# Autodesk Inventor assembly: Estrutura de perfis_999
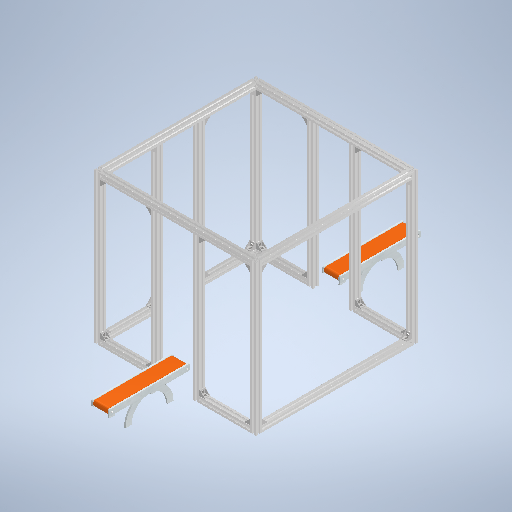
[picture p0: Inventor's stored thumbnail of the model, 512x512]
Saved by Autodesk Inventor 2026 (Build 300175000, 175)
## iProperties
Created: 2025-05-20
Part Number: Estrutura de perfis_999
Document SubType Name: Assembly
Designer: carlo
Author: carlo
## Documents named in this file (11)
- C:\Users\carlo\Documents\Projeto - Braco Robotico\Design\Estrutura de perfis\Estrutura de perfis_999.iam
- C:\Users\carlo\Documents\Projeto - Braco Robotico\Design\Estrutura de perfis\perfil_20x20_001.ipt
- C:\Users\carlo\Documents\Projeto - Braco Robotico\Design\Estrutura de perfis\perfil_20x20_002.ipt
- C:\Users\carlo\Documents\Projeto - Braco Robotico\Design\Estrutura de perfis\perfil_20x20_003.ipt
- C:\Users\carlo\Documents\Projeto - Braco Robotico\Design\Estrutura de perfis\perfil_20x20_004.ipt
- C:\Users\carlo\Documents\Projeto - Braco Robotico\Design\Estrutura de perfis\CBR2020\CBR2020\CBR2020.ipt
- C:\Users\carlo\Documents\Projeto - Braco Robotico\Design\Estrutura de perfis\BPN06M4\BPN06M4\BPN06M4.ipt
- C:\Users\carlo\Documents\Inventor\Content Center Files\R2026\en-US\BS 4183(4)\BS 4183 - M4 x 8(1) III.ipt
- C:\Users\carlo\Documents\Projeto - Braco Robotico\Design\Estrutura de perfis\Conveyor_001_001.ipt
- C:\Users\carlo\Documents\Projeto - Braco Robotico\Design\Estrutura de perfis\Conveyor_002_001.ipt
- C:\Users\carlo\Documents\Projeto - Braco Robotico\Design\Estrutura de perfis\Conveyor_003_001.ipt
## Components (169 placed, 10 different names)
1. perfil_20x20_001:1 — Flush:6, Mate:4, Flush:10
2. perfil_20x20_001:3 — Flush:13, Mate:6, Flush:14, Mate:8, Flush:39, Flush:62
3. perfil_20x20_001:4 — Flush:4, Mate:1, Flush:8, Mate:3, Flush:9, Flush:32
4. perfil_20x20_002:1 — Flush:4, Mate:1, Flush:6, Mate:30
5. perfil_20x20_002:3 — Flush:8, Mate:3, Flush:9, Mate:4, Flush:10, Flush:11, Mate:5, Flush:12, Flush:13, Mate:6, Flush:14, Mate:34, Flush:49, Mate:35, Flush:51
6. perfil_20x20_003:1 — Flush:11, Mate:5, Flush:12, Flush:15, Mate:7, Flush:16, Mate:33, Mate:38
7. perfil_20x20_004:1 — Flush:15, Mate:7, Flush:16, Flush:17, Symmetry:1, Flush:48, Flush:63, Flush:64
8. perfil_20x20_004:2 — Flush:17, Mate:8, Symmetry:1, Flush:18, Mate:9, Flush:19
9. perfil_20x20_003:2 — Flush:18, Mate:9, Flush:19, Flush:20, Mate:10, Flush:21
10. perfil_20x20_002:4 — Flush:20, Mate:10, Flush:21, Flush:22, Mate:11, Flush:23, Flush:24, Flush:31, Mate:23
11. perfil_20x20_001:5 — Flush:22, Mate:11, Flush:23, Mate:12, Flush:25, Mate:25
12. perfil_20x20_002:5 — Flush:24, Mate:12, Flush:25, Mate:24, Flush:38, Mate:28, Flush:40, Mate:29, Flush:44
13. perfil_20x20_003:3 — Flush:31, Flush:32, Mate:23, Flush:33, Flush:34, Flush:35, Mate:26
14. perfil_20x20_003:4 — Flush:33, Mate:24, Flush:34, Mate:27, Flush:41
15. perfil_20x20_004:3 — Flush:35, Mate:25, Mate:26, Flush:36, Flush:37
16. perfil_20x20_004:4 — Flush:36, Flush:37, Mate:27, Flush:45
17. perfil_20x20_001:6 — Flush:38, Flush:39, Mate:28, Flush:57
18. perfil_20x20_003:5 — Flush:40, Flush:41, Mate:29, Flush:42, Flush:43, Mate:31
19. perfil_20x20_003:6 — Flush:42, Flush:43, Mate:30, Mate:32
20. perfil_20x20_004:5 — Flush:44, Flush:45, Mate:31, Flush:46, Flush:47
21. perfil_20x20_004:6 — Flush:46, Flush:47, Mate:32, Flush:58, Flush:59
22. CBR2020:17
23. BPN06M4:33
24. BS 4183 Specification for machine screws and machine screw nuts. Metric series - Metric M4 x 8:33
25. BPN06M4:34
26. BS 4183 Specification for machine screws and machine screw nuts. Metric series - Metric M4 x 8:34
27. CBR2020:18
28. BPN06M4:35
29. BS 4183 Specification for machine screws and machine screw nuts. Metric series - Metric M4 x 8:35
30. BPN06M4:36
31. BS 4183 Specification for machine screws and machine screw nuts. Metric series - Metric M4 x 8:36
32. CBR2020:19
33. BPN06M4:37
34. BS 4183 Specification for machine screws and machine screw nuts. Metric series - Metric M4 x 8:37
35. BPN06M4:38
36. BS 4183 Specification for machine screws and machine screw nuts. Metric series - Metric M4 x 8:38
37. CBR2020:20
38. BPN06M4:39
39. BS 4183 Specification for machine screws and machine screw nuts. Metric series - Metric M4 x 8:39
40. BPN06M4:40
41. BS 4183 Specification for machine screws and machine screw nuts. Metric series - Metric M4 x 8:40
42. CBR2020:21
43. BPN06M4:41
44. BS 4183 Specification for machine screws and machine screw nuts. Metric series - Metric M4 x 8:41
45. BPN06M4:42
46. BS 4183 Specification for machine screws and machine screw nuts. Metric series - Metric M4 x 8:42
47. CBR2020:22
48. BPN06M4:43
49. BS 4183 Specification for machine screws and machine screw nuts. Metric series - Metric M4 x 8:43
50. BPN06M4:44
51. BS 4183 Specification for machine screws and machine screw nuts. Metric series - Metric M4 x 8:44
52. CBR2020:23
53. BPN06M4:45
54. BS 4183 Specification for machine screws and machine screw nuts. Metric series - Metric M4 x 8:45
55. BPN06M4:46
56. BS 4183 Specification for machine screws and machine screw nuts. Metric series - Metric M4 x 8:46
57. CBR2020:24
58. BPN06M4:47
59. BS 4183 Specification for machine screws and machine screw nuts. Metric series - Metric M4 x 8:47
60. BPN06M4:48
61. BS 4183 Specification for machine screws and machine screw nuts. Metric series - Metric M4 x 8:48
62. CBR2020:25
63. BPN06M4:49
64. BS 4183 Specification for machine screws and machine screw nuts. Metric series - Metric M4 x 8:49
65. BPN06M4:50
66. BS 4183 Specification for machine screws and machine screw nuts. Metric series - Metric M4 x 8:50
67. CBR2020:26
68. BPN06M4:51
69. BS 4183 Specification for machine screws and machine screw nuts. Metric series - Metric M4 x 8:51
70. BPN06M4:52
71. BS 4183 Specification for machine screws and machine screw nuts. Metric series - Metric M4 x 8:52
72. CBR2020:27
73. BPN06M4:53
74. BS 4183 Specification for machine screws and machine screw nuts. Metric series - Metric M4 x 8:53
75. BPN06M4:54
76. BS 4183 Specification for machine screws and machine screw nuts. Metric series - Metric M4 x 8:54
77. CBR2020:28
78. BPN06M4:55
79. BS 4183 Specification for machine screws and machine screw nuts. Metric series - Metric M4 x 8:55
80. BPN06M4:56
81. BS 4183 Specification for machine screws and machine screw nuts. Metric series - Metric M4 x 8:56
82. CBR2020:9
83. BPN06M4:17
84. BS 4183 Specification for machine screws and machine screw nuts. Metric series - Metric M4 x 8:17
85. BPN06M4:18
86. BS 4183 Specification for machine screws and machine screw nuts. Metric series - Metric M4 x 8:18
87. CBR2020:10
88. BPN06M4:19
89. BS 4183 Specification for machine screws and machine screw nuts. Metric series - Metric M4 x 8:19
90. BPN06M4:20
91. BS 4183 Specification for machine screws and machine screw nuts. Metric series - Metric M4 x 8:20
92. CBR2020:11
93. BPN06M4:21
94. BS 4183 Specification for machine screws and machine screw nuts. Metric series - Metric M4 x 8:21
95. BPN06M4:22
96. BS 4183 Specification for machine screws and machine screw nuts. Metric series - Metric M4 x 8:22
97. CBR2020:12
98. BPN06M4:23
99. BS 4183 Specification for machine screws and machine screw nuts. Metric series - Metric M4 x 8:23
100. BPN06M4:24
101. BS 4183 Specification for machine screws and machine screw nuts. Metric series - Metric M4 x 8:24
102. CBR2020:13
103. BPN06M4:25
104. BS 4183 Specification for machine screws and machine screw nuts. Metric series - Metric M4 x 8:25
105. BPN06M4:26
106. BS 4183 Specification for machine screws and machine screw nuts. Metric series - Metric M4 x 8:26
107. CBR2020:14
108. BPN06M4:27
109. BS 4183 Specification for machine screws and machine screw nuts. Metric series - Metric M4 x 8:27
110. BPN06M4:28
111. BS 4183 Specification for machine screws and machine screw nuts. Metric series - Metric M4 x 8:28
112. CBR2020:15
113. BPN06M4:29
114. BS 4183 Specification for machine screws and machine screw nuts. Metric series - Metric M4 x 8:29
115. BPN06M4:30
116. BS 4183 Specification for machine screws and machine screw nuts. Metric series - Metric M4 x 8:30
117. CBR2020:16
118. BPN06M4:31
119. BS 4183 Specification for machine screws and machine screw nuts. Metric series - Metric M4 x 8:31
120. BPN06M4:32
121. BS 4183 Specification for machine screws and machine screw nuts. Metric series - Metric M4 x 8:32
122. CBR2020:5
123. BPN06M4:9
124. BS 4183 Specification for machine screws and machine screw nuts. Metric series - Metric M4 x 8:9
125. BPN06M4:10
126. BS 4183 Specification for machine screws and machine screw nuts. Metric series - Metric M4 x 8:10
127. CBR2020:6
128. BPN06M4:11
129. BS 4183 Specification for machine screws and machine screw nuts. Metric series - Metric M4 x 8:11
130. BPN06M4:12
131. BS 4183 Specification for machine screws and machine screw nuts. Metric series - Metric M4 x 8:12
132. CBR2020:7
133. BPN06M4:13
134. BS 4183 Specification for machine screws and machine screw nuts. Metric series - Metric M4 x 8:13
135. BPN06M4:14
136. BS 4183 Specification for machine screws and machine screw nuts. Metric series - Metric M4 x 8:14
137. CBR2020:8
138. BPN06M4:15
139. BS 4183 Specification for machine screws and machine screw nuts. Metric series - Metric M4 x 8:15
140. BPN06M4:16
141. BS 4183 Specification for machine screws and machine screw nuts. Metric series - Metric M4 x 8:16
142. CBR2020:3
143. BPN06M4:5
144. BS 4183 Specification for machine screws and machine screw nuts. Metric series - Metric M4 x 8:5
145. BPN06M4:6
146. BS 4183 Specification for machine screws and machine screw nuts. Metric series - Metric M4 x 8:6
147. CBR2020:4
148. BPN06M4:7
149. BS 4183 Specification for machine screws and machine screw nuts. Metric series - Metric M4 x 8:7
150. BPN06M4:8
151. BS 4183 Specification for machine screws and machine screw nuts. Metric series - Metric M4 x 8:8
152. CBR2020:2
153. BPN06M4:3
154. BS 4183 Specification for machine screws and machine screw nuts. Metric series - Metric M4 x 8:3
155. BPN06M4:4
156. BS 4183 Specification for machine screws and machine screw nuts. Metric series - Metric M4 x 8:4
157. BS 4183 Specification for machine screws and machine screw nuts. Metric series - Metric M4 x 8:2 — Mate:39, Mate:40
158. BPN06M4:2 — Flush:51, Mate:38, Flush:52, Mate:39
159. BS 4183 Specification for machine screws and machine screw nuts. Metric series - Metric M4 x 8:1 — Mate:36, Mate:37
160. BPN06M4:1 — Flush:49, Mate:35, Flush:50, Mate:36
161. CBR2020:1 — Flush:48, Mate:33, Mate:34, Flush:50, Mate:37, Flush:52, Mate:40
162. Conveyor_003_001:1 — Mate:43, Mate:44, Mate:49
163. Conveyor_002_001:2 — Mate:42, Flush:54, Mate:49
164. Conveyor_002_001:1 — Mate:41, Flush:53, Mate:43
165. Conveyor_001_001:1 — Mate:41, Flush:53, Mate:42, Flush:54, Mate:44, Flush:57, Flush:58, Flush:59
166. Conveyor_001_001:2 — Flush:62, Flush:63, Flush:64
167. Conveyor_002_001:3
168. Conveyor_002_001:4
169. Conveyor_003_001:2
## Relationships (92: Flush 52, Mate 39, Symmetry 1)
- Flush:4: perfil_20x20_001:4 ↔ perfil_20x20_002:1
- Mate:1: perfil_20x20_001:4 ↔ perfil_20x20_002:1
- Flush:6: perfil_20x20_001:1 ↔ perfil_20x20_002:1
- Flush:8: perfil_20x20_001:4 ↔ perfil_20x20_002:3
- Mate:3: perfil_20x20_001:4 ↔ perfil_20x20_002:3
- Flush:9: perfil_20x20_001:4 ↔ perfil_20x20_002:3
- Mate:4: perfil_20x20_001:1 ↔ perfil_20x20_002:3
- Flush:10: perfil_20x20_001:1 ↔ perfil_20x20_002:3
- Flush:11: perfil_20x20_002:3 ↔ perfil_20x20_003:1
- Mate:5: perfil_20x20_002:3 ↔ perfil_20x20_003:1
- Flush:12: perfil_20x20_002:3 ↔ perfil_20x20_003:1
- Flush:13: perfil_20x20_001:3 ↔ perfil_20x20_002:3
- Mate:6: perfil_20x20_001:3 ↔ perfil_20x20_002:3
- Flush:14: perfil_20x20_001:3 ↔ perfil_20x20_002:3
- Flush:15: perfil_20x20_003:1 ↔ perfil_20x20_004:1
- Mate:7: perfil_20x20_003:1 ↔ perfil_20x20_004:1
- Flush:16: perfil_20x20_003:1 ↔ perfil_20x20_004:1
- Flush:17: perfil_20x20_004:1 ↔ perfil_20x20_004:2
- Mate:8: perfil_20x20_001:3 ↔ perfil_20x20_004:2
- Symmetry:1: perfil_20x20_004:1 ↔ perfil_20x20_004:2
- Flush:18: perfil_20x20_004:2 ↔ perfil_20x20_003:2
- Mate:9: perfil_20x20_004:2 ↔ perfil_20x20_003:2
- Flush:19: perfil_20x20_004:2 ↔ perfil_20x20_003:2
- Flush:20: perfil_20x20_003:2 ↔ perfil_20x20_002:4
- Mate:10: perfil_20x20_003:2 ↔ perfil_20x20_002:4
- Flush:21: perfil_20x20_003:2 ↔ perfil_20x20_002:4
- Flush:22: perfil_20x20_002:4 ↔ perfil_20x20_001:5
- Mate:11: perfil_20x20_002:4 ↔ perfil_20x20_001:5
- Flush:23: perfil_20x20_002:4 ↔ perfil_20x20_001:5
- Flush:24: perfil_20x20_002:4 ↔ perfil_20x20_002:5
- Mate:12: perfil_20x20_001:5 ↔ perfil_20x20_002:5
- Flush:25: perfil_20x20_001:5 ↔ perfil_20x20_002:5
- Flush:31: perfil_20x20_002:4 ↔ perfil_20x20_003:3
- Flush:32: perfil_20x20_001:4 ↔ perfil_20x20_003:3
- Mate:23: perfil_20x20_002:4 ↔ perfil_20x20_003:3
- Flush:33: perfil_20x20_003:3 ↔ perfil_20x20_003:4
- Mate:24: perfil_20x20_002:5 ↔ perfil_20x20_003:4
- Flush:34: perfil_20x20_003:3 ↔ perfil_20x20_003:4
- Flush:35: perfil_20x20_003:3 ↔ perfil_20x20_004:3
- Mate:25: perfil_20x20_001:5 ↔ perfil_20x20_004:3
- Mate:26: perfil_20x20_003:3 ↔ perfil_20x20_004:3
- Flush:36: perfil_20x20_004:3 ↔ perfil_20x20_004:4
- Flush:37: perfil_20x20_004:3 ↔ perfil_20x20_004:4
- Mate:27: perfil_20x20_003:4 ↔ perfil_20x20_004:4
- Flush:38: perfil_20x20_002:5 ↔ perfil_20x20_001:6
- Flush:39: perfil_20x20_001:3 ↔ perfil_20x20_001:6
- Mate:28: perfil_20x20_002:5 ↔ perfil_20x20_001:6
- Flush:40: perfil_20x20_002:5 ↔ perfil_20x20_003:5
- Flush:41: perfil_20x20_003:4 ↔ perfil_20x20_003:5
- Mate:29: perfil_20x20_002:5 ↔ perfil_20x20_003:5
- Flush:42: perfil_20x20_003:5 ↔ perfil_20x20_003:6
- Flush:43: perfil_20x20_003:5 ↔ perfil_20x20_003:6
- Mate:30: perfil_20x20_002:1 ↔ perfil_20x20_003:6
- Flush:44: perfil_20x20_002:5 ↔ perfil_20x20_004:5
- Flush:45: perfil_20x20_004:4 ↔ perfil_20x20_004:5
- Mate:31: perfil_20x20_003:5 ↔ perfil_20x20_004:5
- Flush:46: perfil_20x20_004:5 ↔ perfil_20x20_004:6
- Flush:47: perfil_20x20_004:5 ↔ perfil_20x20_004:6
- Mate:32: perfil_20x20_003:6 ↔ perfil_20x20_004:6
- Flush:48: perfil_20x20_004:1 ↔ CBR2020:1
- Mate:33: perfil_20x20_003:1 ↔ CBR2020:1
- Mate:34: perfil_20x20_002:3 ↔ CBR2020:1
- Flush:49: perfil_20x20_002:3 ↔ BPN06M4:1
- Mate:35: perfil_20x20_002:3 ↔ BPN06M4:1
- Flush:50: BPN06M4:1 ↔ CBR2020:1
- Mate:36: BS 4183 Specification for machine screws and machine screw nuts. Metric series - Metric M4 x 8:1 ↔ BPN06M4:1
- Mate:37: BS 4183 Specification for machine screws and machine screw nuts. Metric series - Metric M4 x 8:1 ↔ CBR2020:1
- Flush:51: perfil_20x20_002:3 ↔ BPN06M4:2
- Mate:38: perfil_20x20_003:1 ↔ BPN06M4:2
- Flush:52: BPN06M4:2 ↔ CBR2020:1
- Mate:39: BS 4183 Specification for machine screws and machine screw nuts. Metric series - Metric M4 x 8:2 ↔ BPN06M4:2
- Mate:40: BS 4183 Specification for machine screws and machine screw nuts. Metric series - Metric M4 x 8:2 ↔ CBR2020:1
- Mate:41: Conveyor_002_001:1 ↔ Conveyor_001_001:1
- Flush:53 (-2.5 mm): Conveyor_002_001:1 ↔ Conveyor_001_001:1
- Mate:42: Conveyor_002_001:2 ↔ Conveyor_001_001:1
- Flush:54 (-2.5 mm): Conveyor_002_001:2 ↔ Conveyor_001_001:1
- Mate:43: Conveyor_003_001:1 ↔ Conveyor_002_001:1
- Mate:44 (1 mm): Conveyor_003_001:1 ↔ Conveyor_001_001:1
- Flush:57: perfil_20x20_001:6 ↔ Conveyor_001_001:1
- Flush:58: perfil_20x20_004:6 ↔ Conveyor_001_001:1
- Mate:49: Conveyor_003_001:1 ↔ Conveyor_002_001:2
- Flush:59: perfil_20x20_004:6 ↔ Conveyor_001_001:1
- [Mate]: Conveyor_001_001:2 ↔ Conveyor_002_001:3
- [Flush] (-2.5 mm): Conveyor_001_001:2 ↔ Conveyor_002_001:3
- [Mate]: Conveyor_001_001:2 ↔ Conveyor_002_001:4
- [Flush] (-2.5 mm): Conveyor_001_001:2 ↔ Conveyor_002_001:4
- [Mate]: Conveyor_002_001:3 ↔ Conveyor_003_001:2
- [Mate] (1 mm): Conveyor_001_001:2 ↔ Conveyor_003_001:2
- [Mate]: Conveyor_002_001:4 ↔ Conveyor_003_001:2
- Flush:62: perfil_20x20_001:3 ↔ Conveyor_001_001:2
- Flush:63: perfil_20x20_004:1 ↔ Conveyor_001_001:2
- Flush:64: perfil_20x20_004:1 ↔ Conveyor_001_001:2
## Named parameters: d245_d234 = 1 mm, d246_d243 = 0 mm, d247_d229 = 0 mm, d248_d230 = -2.5 mm, d249_d231 = 0 mm, d250_d232 = -2.5 mm, d251_d233 = 0 mm
